# Autodesk Inventor assembly: plotter
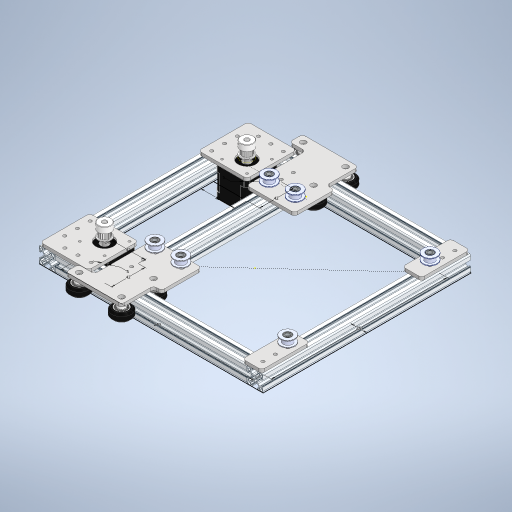
[picture p0: Inventor's stored thumbnail of the model, 512x512]
Saved by Autodesk Inventor 2023.1 (Build 271208000, 208)
## iProperties
Created: 2025-11-24
Part Number: plotter
Document SubType Name: Assembly
Designer: DELL
Author: DELL
## Documents named in this file (18)
- C:\Users\DELL\reposGitHub\VSOSH25-26\models\plotter\plotter.iam
- C:\Users\DELL\reposGitHub\VSOSH25-26\models\plotter\эскиз.ipt
- C:\Users\DELL\reposGitHub\VSOSH25-26\models\import\222LX-Konstruktsionnyy-profil-20kh20L.ipt
- C:\Users\DELL\reposGitHub\VSOSH25-26\models\plotter\профиль2020.ipt
- C:\Users\DELL\reposGitHub\VSOSH25-26\models\import\Schrittmotor-42SHDC3025-24B.ipt
- C:\Users\DELL\reposGitHub\VSOSH25-26\models\plotter\креп_мотора.ipt
- C:\Users\DELL\reposGitHub\VSOSH25-26\models\plotter\креп_мотора_MIR.ipt
- C:\Users\DELL\reposGitHub\VSOSH25-26\models\import\profil.ipt
- C:\Users\DELL\reposGitHub\VSOSH25-26\models\plotter\креп_центр_рейки.ipt
- C:\Users\DELL\reposGitHub\VSOSH25-26\models\import\V-ролик сборка.ipt
- C:\Users\DELL\reposGitHub\VSOSH25-26\models\import\Ролик с резьбой GT2 на моторы.ipt
- C:\Users\DELL\reposGitHub\VSOSH25-26\models\import\Сборка ролик с подшипником.ipt
- C:\Users\DELL\reposGitHub\VSOSH25-26\models\plotter\креп_центр_рейки_MIR1.ipt
- C:\Users\DELL\reposGitHub\VSOSH25-26\models\import\V-ролик сборка_MIR1.ipt
- C:\Users\DELL\reposGitHub\VSOSH25-26\models\plotter\креп. пасс. ролика.ipt
- C:\Users\DELL\reposGitHub\VSOSH25-26\models\import\Ролик с резьбой GT2 на моторы_MIR.ipt
- C:\Users\DELL\reposGitHub\VSOSH25-26\models\import\Сборка ролик с подшипником_MIR1.ipt
- C:\Users\DELL\reposGitHub\VSOSH25-26\models\plotter\креп. пасс. ролика_MIR.ipt
## Components (28 placed, 19 different names)
1. эскиз:1
2. профиль24Левый — Совмещение:10, Заподлицо:2, Совмещение:12, Заподлицо:3, Совмещение:13, Совмещение:15, Совмещение:16, Совмещение:19, Совмещение:23, Совмещение:28, Совмещение:61
3. профиль24правый — Совмещение:1, Заподлицо:1, Совмещение:11, Совмещение:17, Совмещение:18, Совмещение:22, Совмещение:37, Заподлицо:9
4. профиль16Верх:1 — Заподлицо:1, Совмещение:11, Заподлицо:2, Совмещение:12, Совмещение:15, Совмещение:17, Совмещение:20, Заподлицо:5
5. профиь26низ — Заподлицо:3, Совмещение:13, Совмещение:16, Совмещение:18, Заподлицо:4, Совмещение:21, Совмещение:24
6. Schrittmotor-42SHDC3025-24B:1 — Заподлицо:4, Совмещение:21, Совмещение:22, Заподлицо:6, Совмещение:38
7. Schrittmotor-42SHDC3025-24B:2 — Заподлицо:5, Совмещение:23, Совмещение:24
8. креп_мотора:1 — Заподлицо:6
9. креп_мотора_MIR:1
10. profil:1 — Совмещение:25, Совмещение:28, Заподлицо:8
11. креп_центр_рейки:1 — Совмещение:29, Совмещение:30, Совмещение:31, Совмещение:32, Совмещение:33, Совмещение:34, Совмещение:37, Заподлицо:7, Совмещение:40, Совмещение:62, Заподлицо:8, Совмещение:63, Совмещение:64, Совмещение:65
12. V-ролик сборка:1 — Совмещение:29, Совмещение:30
13. V-ролик сборка:2 — Совмещение:31, Совмещение:32
14. V-ролик сборка:3 — Совмещение:33, Совмещение:34
15. Ролик с резьбой GT2 на моторы:1 — Совмещение:38
16. Сборка ролик с подшипником:1 — Совмещение:40, Совмещение:62
17. креп_центр_рейки_MIR1:1 — Совмещение:54, Совмещение:55, Совмещение:56, Совмещение:57, Совмещение:58, Совмещение:59, Совмещение:60, Совмещение:61
18. V-ролик сборка_MIR1:1 — Совмещение:55, Совмещение:56
19. V-ролик сборка_MIR1:2 — Совмещение:57, Совмещение:58
20. V-ролик сборка_MIR1:3 — Совмещение:59, Совмещение:60
21. Сборка ролик с подшипником:2 — Совмещение:63, Совмещение:64, Совмещение:65
22. креп. пасс. ролика:1 — Заподлицо:9, Совмещение:66, Совмещение:67
23. Сборка ролик с подшипником:3 — Совмещение:66, Совмещение:67
24. Ролик с резьбой GT2 на моторы_MIR:1
25. Сборка ролик с подшипником_MIR1:1
26. Сборка ролик с подшипником_MIR1:2
27. креп. пасс. ролика_MIR:1 — Совмещение:68, Совмещение:69
28. Сборка ролик с подшипником_MIR1:3 — Совмещение:68, Совмещение:69
## Relationships (51: Mate 42, Flush 9)
- Совмещение:1 [Mate]: профиль24правый
- Совмещение:10 [Mate]: профиль24Левый
- Заподлицо:1 [Flush]: профиль24правый ↔ профиль16Верх:1
- Совмещение:11 [Mate]: профиль24правый ↔ профиль16Верх:1
- Заподлицо:2 [Flush]: профиль24Левый ↔ профиль16Верх:1
- Совмещение:12 [Mate]: профиль24Левый ↔ профиль16Верх:1
- Заподлицо:3 [Flush]: профиль24Левый ↔ профиь26низ
- Совмещение:13 [Mate]: профиль24Левый ↔ профиь26низ
- Совмещение:15 [Mate]: профиль24Левый ↔ профиль16Верх:1
- Совмещение:16 [Mate]: профиль24Левый ↔ профиь26низ
- Совмещение:17 [Mate]: профиль24правый ↔ профиль16Верх:1
- Совмещение:18 [Mate]: профиль24правый ↔ профиь26низ
- Совмещение:19 [Mate] (110 mm): профиль24Левый
- Совмещение:20 [Mate] (120 mm): профиль16Верх:1
- Заподлицо:4 [Flush]: профиь26низ ↔ Schrittmotor-42SHDC3025-24B:1
- Совмещение:21 [Mate]: профиь26низ ↔ Schrittmotor-42SHDC3025-24B:1
- Совмещение:22 [Mate]: профиль24правый ↔ Schrittmotor-42SHDC3025-24B:1
- Заподлицо:5 [Flush]: профиль16Верх:1 ↔ Schrittmotor-42SHDC3025-24B:2
- Совмещение:23 [Mate]: профиль24Левый ↔ Schrittmotor-42SHDC3025-24B:2
- Совмещение:24 [Mate]: профиь26низ ↔ Schrittmotor-42SHDC3025-24B:2
- Заподлицо:6 [Flush]: Schrittmotor-42SHDC3025-24B:1 ↔ креп_мотора:1
- Совмещение:25 [Mate]: profil:1
- Совмещение:28 [Mate] (10 mm): профиль24Левый ↔ profil:1
- Совмещение:29 [Mate]: креп_центр_рейки:1 ↔ V-ролик сборка:1
- Совмещение:30 [Mate]: креп_центр_рейки:1 ↔ V-ролик сборка:1
- Совмещение:31 [Mate]: креп_центр_рейки:1 ↔ V-ролик сборка:2
- Совмещение:32 [Mate]: креп_центр_рейки:1 ↔ V-ролик сборка:2
- Совмещение:33 [Mate]: креп_центр_рейки:1 ↔ V-ролик сборка:3
- Совмещение:34 [Mate]: креп_центр_рейки:1 ↔ V-ролик сборка:3
- Совмещение:37 [Mate] (2 mm): профиль24правый ↔ креп_центр_рейки:1
- Заподлицо:7 [Flush] (-58.5 mm): креп_центр_рейки:1
- Совмещение:38 [Mate]: Schrittmotor-42SHDC3025-24B:1 ↔ Ролик с резьбой GT2 на моторы:1
- Совмещение:40 [Mate] (5 mm): креп_центр_рейки:1 ↔ Сборка ролик с подшипником:1
- Совмещение:54 [Mate] (58.5 mm): креп_центр_рейки_MIR1:1
- Совмещение:55 [Mate]: креп_центр_рейки_MIR1:1 ↔ V-ролик сборка_MIR1:1
- Совмещение:56 [Mate]: креп_центр_рейки_MIR1:1 ↔ V-ролик сборка_MIR1:1
- Совмещение:57 [Mate]: креп_центр_рейки_MIR1:1 ↔ V-ролик сборка_MIR1:2
- Совмещение:58 [Mate]: креп_центр_рейки_MIR1:1 ↔ V-ролик сборка_MIR1:2
- Совмещение:59 [Mate]: креп_центр_рейки_MIR1:1 ↔ V-ролик сборка_MIR1:3
- Совмещение:60 [Mate]: креп_центр_рейки_MIR1:1 ↔ V-ролик сборка_MIR1:3
- Совмещение:61 [Mate] (2 mm): профиль24Левый ↔ креп_центр_рейки_MIR1:1
- Совмещение:62 [Mate]: креп_центр_рейки:1 ↔ Сборка ролик с подшипником:1
- Заподлицо:8 [Flush] (5.5 mm): profil:1 ↔ креп_центр_рейки:1
- Совмещение:63 [Mate]: креп_центр_рейки:1 ↔ Сборка ролик с подшипником:2
- Совмещение:64 [Mate] (5 mm): креп_центр_рейки:1 ↔ Сборка ролик с подшипником:2
- Совмещение:65 [Mate]: креп_центр_рейки:1 ↔ Сборка ролик с подшипником:2
- Заподлицо:9 [Flush]: профиль24правый ↔ креп. пасс. ролика:1
- Совмещение:66 [Mate] (5 mm): креп. пасс. ролика:1 ↔ Сборка ролик с подшипником:3
- Совмещение:67 [Mate]: креп. пасс. ролика:1 ↔ Сборка ролик с подшипником:3
- Совмещение:68 [Mate]: креп. пасс. ролика_MIR:1 ↔ Сборка ролик с подшипником_MIR1:3
- Совмещение:69 [Mate] (5 mm): креп. пасс. ролика_MIR:1 ↔ Сборка ролик с подшипником_MIR1:3
